# Autodesk Inventor assembly: Сборка1
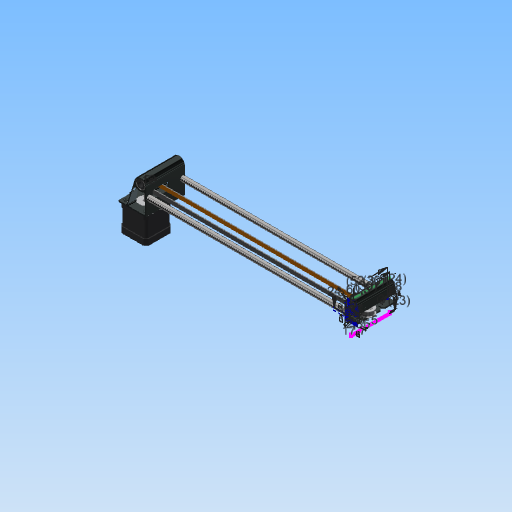
[picture p0: Inventor's stored thumbnail of the model, 512x512]
Saved by Autodesk Inventor 2017 (Build 210142000, 142)
## iProperties
Part Number: Сборка1
Material: Типовые
Document SubType Name: Assembly
Designer: Max
Author: Max
## Documents named in this file (10)
- C:\Users\Max\Desktop\Flying Bear Ghost 5\y-axis.iam
- C:\Users\Max\Desktop\Flying Bear Ghost 5\screw m3.ipt
- C:\Users\Max\Desktop\Flying Bear Ghost 5\2GT 5mm 0.ipt
- C:\Users\Max\Desktop\Flying Bear Ghost 5\2GT 5mm 2.ipt
- C:\Users\Max\Desktop\Flying Bear Ghost 5\linear bearing 8x15x24.ipt
- C:\Users\Max\Desktop\Flying Bear Ghost 5\LEFT CARRIAGE.ipt
- C:\Users\Max\Desktop\Flying Bear Ghost 5\42-40.ipt
- C:\Users\Max\Desktop\Flying Bear Ghost 5\Right carriage y.ipt
- C:\Users\Max\Desktop\Flying Bear Ghost 5\shaft 8mm x axis.ipt
- C:\Users\Max\Desktop\Flying Bear Ghost 5\belt x axis.ipt
## Components (21 placed, 9 different names)
1. linear bearing 8x15x24:1 — Заподлицо:90
2. linear bearing 8x15x24:2 — Совмещение:218, Заподлицо:89
3. LEFT CARRIAGE:1 — Совмещение:209, Совмещение:210, Совмещение:211, Совмещение:212, Совмещение:213, Совмещение:214, Совмещение:215, Совмещение:216, Совмещение:218, Заподлицо:89, Заподлицо:90, Заподлицо:93, Совмещение:227
4. 42-40:1 — Совмещение:209, Совмещение:210, Совмещение:211, Совмещение:217, Заподлицо:88
5. screw m3:29 — Совмещение:212, Заподлицо:87
6. screw m3:30 — Совмещение:214, Заподлицо:85, Заподлицо:86
7. screw m3:31 — Совмещение:215, Совмещение:216, Заподлицо:85
8. screw m3:32 — Совмещение:213, Заподлицо:86, Заподлицо:87
9. 2GT 5mm 2:2 — Совмещение:217, Заподлицо:88, Совмещение:237, Совмещение:238
10. Right carriage y:1 — Совмещение:219, Совмещение:220, Заподлицо:91, Заподлицо:92, Заподлицо:93, Совмещение:222, Совмещение:223, Совмещение:224, Совмещение:225, Совмещение:229, Совмещение:230, Совмещение:231, Совмещение:232, Совмещение:233, Совмещение:234, Совмещение:235
11. linear bearing 8x15x24:3 — Совмещение:219, Заподлицо:91
12. linear bearing 8x15x24:4 — Совмещение:220, Заподлицо:92
13. shaft 8mm x axis:1 — Совмещение:222, Совмещение:224, Совмещение:226
14. shaft 8mm x axis:2 — Совмещение:223, Совмещение:225, Совмещение:228
15. screw m3:33 — Совмещение:226, Совмещение:227, Заподлицо:94
16. screw m3:34 — Совмещение:228, Заподлицо:94
17. screw m3:35 — Совмещение:229, Заподлицо:95
18. screw m3:36 — Совмещение:230, Заподлицо:95, Совмещение:231
19. 2GT 5mm 0:4 — Совмещение:232, Совмещение:235, Совмещение:236
20. screw m3:37 — Совмещение:233, Совмещение:234
21. belt x axis:1 — Совмещение:236, Совмещение:237, Совмещение:238
## Relationships (40: Mate 29, Flush 11)
- Совмещение:209 [Mate]: LEFT CARRIAGE:1 ↔ 42-40:1
- Совмещение:210 [Mate]: LEFT CARRIAGE:1 ↔ 42-40:1
- Совмещение:211 [Mate]: LEFT CARRIAGE:1 ↔ 42-40:1
- Совмещение:212 [Mate]: LEFT CARRIAGE:1 ↔ screw m3:29
- Совмещение:213 [Mate]: LEFT CARRIAGE:1 ↔ screw m3:32
- Совмещение:214 [Mate]: LEFT CARRIAGE:1 ↔ screw m3:30
- Совмещение:215 [Mate]: LEFT CARRIAGE:1 ↔ screw m3:31
- Совмещение:216 [Mate]: LEFT CARRIAGE:1 ↔ screw m3:31
- Заподлицо:85 [Flush]: screw m3:30 ↔ screw m3:31
- Заподлицо:86 [Flush]: screw m3:30 ↔ screw m3:32
- Заподлицо:87 [Flush]: screw m3:29 ↔ screw m3:32
- Совмещение:217 [Mate]: 42-40:1 ↔ 2GT 5mm 2:2
- Заподлицо:88 [Flush] (0.5 mm): 42-40:1 ↔ 2GT 5mm 2:2
- Совмещение:218 [Mate]: linear bearing 8x15x24:2 ↔ LEFT CARRIAGE:1
- Заподлицо:89 [Flush]: linear bearing 8x15x24:2 ↔ LEFT CARRIAGE:1
- Заподлицо:90 [Flush]: linear bearing 8x15x24:1 ↔ LEFT CARRIAGE:1
- Совмещение:219 [Mate]: Right carriage y:1 ↔ linear bearing 8x15x24:3
- Совмещение:220 [Mate]: Right carriage y:1 ↔ linear bearing 8x15x24:4
- Заподлицо:91 [Flush]: Right carriage y:1 ↔ linear bearing 8x15x24:3
- Заподлицо:92 [Flush]: Right carriage y:1 ↔ linear bearing 8x15x24:4
- Заподлицо:93 [Flush]: LEFT CARRIAGE:1 ↔ Right carriage y:1
- Совмещение:222 [Mate]: Right carriage y:1 ↔ shaft 8mm x axis:1
- Совмещение:223 [Mate]: Right carriage y:1 ↔ shaft 8mm x axis:2
- Совмещение:224 [Mate]: Right carriage y:1 ↔ shaft 8mm x axis:1
- Совмещение:225 [Mate]: Right carriage y:1 ↔ shaft 8mm x axis:2
- Совмещение:226 [Mate]: shaft 8mm x axis:1 ↔ screw m3:33
- Совмещение:227 [Mate]: LEFT CARRIAGE:1 ↔ screw m3:33
- Совмещение:228 [Mate]: shaft 8mm x axis:2 ↔ screw m3:34
- Заподлицо:94 [Flush]: screw m3:33 ↔ screw m3:34
- Совмещение:229 [Mate]: Right carriage y:1 ↔ screw m3:35
- Совмещение:230 [Mate]: Right carriage y:1 ↔ screw m3:36
- Заподлицо:95 [Flush]: screw m3:35 ↔ screw m3:36
- Совмещение:231 [Mate]: Right carriage y:1 ↔ screw m3:36
- Совмещение:232 [Mate]: Right carriage y:1 ↔ 2GT 5mm 0:4
- Совмещение:233 [Mate]: Right carriage y:1 ↔ screw m3:37
- Совмещение:234 [Mate]: Right carriage y:1 ↔ screw m3:37
- Совмещение:235 [Mate] (1 mm): Right carriage y:1 ↔ 2GT 5mm 0:4
- Совмещение:236 [Mate]: 2GT 5mm 0:4 ↔ belt x axis:1
- Совмещение:237 [Mate]: 2GT 5mm 2:2 ↔ belt x axis:1
- Совмещение:238 [Mate] (0.3 mm): 2GT 5mm 2:2 ↔ belt x axis:1
